# Autodesk Inventor assembly: Ensamble del Sistema de Balanceo
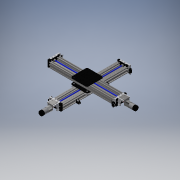
[picture p0: Inventor's stored thumbnail of the model, 180x180]
Saved by Autodesk Inventor 2018.3 (Build 223284000, 284)
## iProperties
Created: 2020-12-03
Part Number: Ensamble del Sistema de Balanceo
Material: Genérico
Description: STEP AP203
Document SubType Name: Assembly
Designer: SERGIO ROMO
Sending System: SolidWorks 2019
Preprocessor: SwSTEP 2.0
Title: Ensamble del Arreglo.STEP
Revision Number: ANY
## Documents named in this file (17)
- C:\Users\SERGIO ROMO\Documents\GitHub\RemBot\CAD\Balanceo de masa\Inventor\Ensamble del Sistema de Balanceo.iam
- C:\Users\SERGIO ROMO\Documents\GitHub\RemBot\CAD\Balanceo de masa\Inventor\C-Beam Actuator Lineal 500mm (Sin motor, sin carrito).ipt
- C:\Users\SERGIO ROMO\Documents\GitHub\RemBot\CAD\Balanceo de masa\Inventor\XLarge C-Beam Gantry Kit.iam
- C:\Users\SERGIO ROMO\Documents\GitHub\RemBot\CAD\Balanceo de masa\Inventor\Clavo.ipt
- C:\Users\SERGIO ROMO\Documents\GitHub\RemBot\CAD\Balanceo de masa\Inventor\Gearmotor_37D_19a1.ipt
- C:\Users\SERGIO ROMO\Documents\GitHub\RemBot\CAD\Balanceo de masa\Inventor\Impresion3D.ipt
- C:\Users\SERGIO ROMO\Documents\GitHub\RemBot\CAD\Balanceo de masa\Inventor\C-Beam Gantry Plate XLarge.step.ipt
- C:\Users\SERGIO ROMO\Documents\GitHub\RemBot\CAD\Balanceo de masa\Inventor\Bracket Inventor.ipt
- C:\Users\SERGIO ROMO\Documents\GitHub\RemBot\CAD\Balanceo de masa\Inventor\KW8-2.ipt
- C:\Users\SERGIO ROMO\Documents\GitHub\RemBot\CAD\Balanceo de masa\Inventor\Impresion3D sin Bracket.ipt
- C:\Users\SERGIO ROMO\Documents\GitHub\RemBot\CAD\Balanceo de masa\Inventor\Clavo de Arriba.ipt
- C:\Users\SERGIO ROMO\Documents\GitHub\RemBot\CAD\Balanceo de masa\Inventor\Tornillo final de carrera.ipt
- C:\Users\SERGIO ROMO\Documents\GitHub\RemBot\CAD\Balanceo de masa\Inventor\Triangulo.ipt
- C:\Users\SERGIO ROMO\Documents\GitHub\RemBot\CAD\Balanceo de masa\Inventor\TornilloM6.ipt
- C:\Users\SERGIO ROMO\Documents\GitHub\RemBot\CAD\Balanceo de masa\Inventor\Tuerca para tornilloM6.ipt
- C:\Users\SERGIO ROMO\Documents\GitHub\RemBot\CAD\Balanceo de masa\Inventor\Tornillo para Bracket.ipt
- C:\Users\SERGIO ROMO\Documents\GitHub\RemBot\CAD\Balanceo de masa\Inventor\Tornillo para Motor Pololu.ipt
## Components (68 placed, 21 different names)
1. C-Beam Actuator Lineal 500mm (Sin motor, sin carrito)_1 — Coincidencia:6, Coincidencia:7, Coincidencia:8, Coincidencia:39, Coincidencia:41, Coincidencia:42, Coincidencia:45
2. XLarge C-Beam Gantry Kit_2 [sub-assembly] — Rígido:1
3. Clavo_8
4. Clavo_9
5. Gearmotor_37D_19a1_10 — Coincidencia:6
6. Gearmotor_37D_19a1_22
7. Impresion3D_28 — Coincidencia:1, Coincidencia:4, Coincidencia:15, Coincidencia:16, Coincidencia:28, Coincidencia:29, Coincidencia:30, Coincidencia:31, Coincidencia:83, Coincidencia:84
8. C-Beam Actuator Lineal 500mm (Sin motor, sin carrito):2 — Rígido:1, Coincidencia:2, Coincidencia:9, Coincidencia:10
9. C-Beam Gantry Plate XLarge.step:1
10. Bracket Inventor:1 — Coincidencia:1, Coincidencia:83, Coincidencia:84, Coincidencia:106, Coincidencia:107, Coincidencia:108, Coincidencia:109, Coincidencia:110, Coincidencia:111, Coincidencia:112, Coincidencia:113, Coincidencia:134, Coincidencia:135, Coincidencia:136, Coincidencia:137, Coincidencia:138, Coincidencia:139, Coincidencia:140, Coincidencia:141, Coincidencia:142, Coincidencia:143, Coincidencia:144, Coincidencia:145
11. Bracket Inventor:2 — Coincidencia:3, Coincidencia:11, Coincidencia:12, Coincidencia:85, Coincidencia:114, Coincidencia:115, Coincidencia:116, Coincidencia:117, Coincidencia:118, Coincidencia:119, Coincidencia:120, Coincidencia:121, Coincidencia:122, Coincidencia:123, Coincidencia:124, Coincidencia:125, Coincidencia:126, Coincidencia:127, Coincidencia:128, Coincidencia:129, Coincidencia:130, Coincidencia:131, Coincidencia:132, Coincidencia:133
12. Impresion3D:2 — Coincidencia:2, Coincidencia:3, Coincidencia:5, Coincidencia:11, Coincidencia:12, Coincidencia:13, Coincidencia:14, Coincidencia:24, Coincidencia:25, Coincidencia:26, Coincidencia:27, Coincidencia:85, Coincidencia:90, Coincidencia:91, Coincidencia:92, Coincidencia:93
13. KW8-2:1 — Coincidencia:4
14. KW8-2:2 — Coincidencia:5
15. KW8-2:3
16. KW8-2:4
17. Impresion3D sin Bracket:1 — Coincidencia:7, Coincidencia:8, Coincidencia:17, Coincidencia:18, Coincidencia:19, Coincidencia:86, Coincidencia:87, Coincidencia:88, Coincidencia:89
18. Impresion3D sin Bracket:2 — Coincidencia:9, Coincidencia:10, Coincidencia:20, Coincidencia:21, Coincidencia:22, Coincidencia:23, Coincidencia:94, Coincidencia:95, Coincidencia:96, Coincidencia:97
19. Clavo:3 — Coincidencia:13
20. Clavo:4 — Coincidencia:14
21. Clavo de Arriba:1 — Coincidencia:15
22. Clavo de Arriba:2 — Coincidencia:16
23. Clavo de Arriba:3 — Coincidencia:17
24. Clavo de Arriba:4 — Coincidencia:18, Coincidencia:19
25. Clavo de Arriba:5 — Coincidencia:21, Coincidencia:23
26. Clavo de Arriba:6 — Coincidencia:20, Coincidencia:22
27. Clavo de Arriba:7 — Coincidencia:24, Coincidencia:25
28. Clavo de Arriba:8 — Coincidencia:26, Coincidencia:27
29. Tornillo final de carrera:1 — Coincidencia:28, Coincidencia:30
30. Tornillo final de carrera:2 — Coincidencia:29, Coincidencia:31
31. Triangulo:1 — Coincidencia:41, Coincidencia:102, Coincidencia:104
32. Triangulo:2 — Coincidencia:42, Coincidencia:98, Coincidencia:100
33. Triangulo:3 — Coincidencia:39, Coincidencia:103, Coincidencia:105
34. Triangulo:4 — Coincidencia:45, Coincidencia:99, Coincidencia:101
35. Tornillo final de carrera:3 — Coincidencia:86, Coincidencia:88
36. Tornillo final de carrera:4 — Coincidencia:87, Coincidencia:89
37. Tornillo final de carrera:5 — Coincidencia:90, Coincidencia:92
38. Tornillo final de carrera:6 — Coincidencia:91, Coincidencia:93
39. Tornillo final de carrera:7 — Coincidencia:94, Coincidencia:96
40. Tornillo final de carrera:8 — Coincidencia:95, Coincidencia:97
41. TornilloM6:5 — Coincidencia:98
42. TornilloM6:6 — Coincidencia:99
43. Tuerca para tornilloM6:5 — Coincidencia:100
44. Tuerca para tornilloM6:6 — Coincidencia:101
45. TornilloM6:7 — Coincidencia:102
46. TornilloM6:8 — Coincidencia:103
47. Tuerca para tornilloM6:7 — Coincidencia:105
48. Tuerca para tornilloM6:8 — Coincidencia:104
49. Tornillo para Bracket:1 — Coincidencia:107, Coincidencia:111
50. Tornillo para Bracket:2 — Coincidencia:108, Coincidencia:112
51. Tornillo para Bracket:3 — Coincidencia:109, Coincidencia:110
52. Tornillo para Bracket:4 — Coincidencia:106, Coincidencia:113
53. Tornillo para Bracket:5 — Coincidencia:116, Coincidencia:121
54. Tornillo para Bracket:6 — Coincidencia:115, Coincidencia:118
55. Tornillo para Bracket:7 — Coincidencia:117, Coincidencia:120
56. Tornillo para Bracket:8 — Coincidencia:114, Coincidencia:119
57. Tornillo para Motor Pololu:1 — Coincidencia:127, Coincidencia:130
58. Tornillo para Motor Pololu:2 — Coincidencia:126, Coincidencia:128
59. Tornillo para Motor Pololu:3 — Coincidencia:124, Coincidencia:132
60. Tornillo para Motor Pololu:4 — Coincidencia:123, Coincidencia:131
61. Tornillo para Motor Pololu:5 — Coincidencia:125, Coincidencia:129
62. Tornillo para Motor Pololu:6 — Coincidencia:122, Coincidencia:133
63. Tornillo para Motor Pololu:7 — Coincidencia:138, Coincidencia:144
64. Tornillo para Motor Pololu:8 — Coincidencia:137, Coincidencia:143
65. Tornillo para Motor Pololu:9 — Coincidencia:136, Coincidencia:145
66. Tornillo para Motor Pololu:10 — Coincidencia:134, Coincidencia:141
67. Tornillo para Motor Pololu:11 — Coincidencia:135, Coincidencia:140
68. Tornillo para Motor Pololu:12 — Coincidencia:139, Coincidencia:142
## Relationships (99: Mate 98, WeldJoint 1)
- Rígido:1 [WeldJoint]: XLarge C-Beam Gantry Kit_2 ↔ C-Beam Actuator Lineal 500mm (Sin motor, sin carrito):2
- Coincidencia:1 [Mate]: Impresion3D_28 ↔ Bracket Inventor:1
- Coincidencia:2 [Mate]: C-Beam Actuator Lineal 500mm (Sin motor, sin carrito):2 ↔ Impresion3D:2
- Coincidencia:3 [Mate]: Bracket Inventor:2 ↔ Impresion3D:2
- Coincidencia:4 [Mate]: Impresion3D_28 ↔ KW8-2:1
- Coincidencia:5 [Mate]: Impresion3D:2 ↔ KW8-2:2
- Coincidencia:6 [Mate]: C-Beam Actuator Lineal 500mm (Sin motor, sin carrito)_1 ↔ Gearmotor_37D_19a1_10
- Coincidencia:7 [Mate]: C-Beam Actuator Lineal 500mm (Sin motor, sin carrito)_1 ↔ Impresion3D sin Bracket:1
- Coincidencia:8 [Mate]: C-Beam Actuator Lineal 500mm (Sin motor, sin carrito)_1 ↔ Impresion3D sin Bracket:1
- Coincidencia:9 [Mate]: C-Beam Actuator Lineal 500mm (Sin motor, sin carrito):2 ↔ Impresion3D sin Bracket:2
- Coincidencia:10 [Mate]: C-Beam Actuator Lineal 500mm (Sin motor, sin carrito):2 ↔ Impresion3D sin Bracket:2
- Coincidencia:11 [Mate]: Bracket Inventor:2 ↔ Impresion3D:2
- Coincidencia:12 [Mate]: Bracket Inventor:2 ↔ Impresion3D:2
- Coincidencia:13 [Mate]: Impresion3D:2 ↔ Clavo:3
- Coincidencia:14 [Mate]: Impresion3D:2 ↔ Clavo:4
- Coincidencia:15 [Mate]: Impresion3D_28 ↔ Clavo de Arriba:1
- Coincidencia:16 [Mate]: Impresion3D_28 ↔ Clavo de Arriba:2
- Coincidencia:17 [Mate]: Impresion3D sin Bracket:1 ↔ Clavo de Arriba:3
- Coincidencia:18 [Mate]: Impresion3D sin Bracket:1 ↔ Clavo de Arriba:4
- Coincidencia:19 [Mate]: Impresion3D sin Bracket:1 ↔ Clavo de Arriba:4
- Coincidencia:20 [Mate]: Impresion3D sin Bracket:2 ↔ Clavo de Arriba:6
- Coincidencia:21 [Mate]: Impresion3D sin Bracket:2 ↔ Clavo de Arriba:5
- Coincidencia:22 [Mate]: Impresion3D sin Bracket:2 ↔ Clavo de Arriba:6
- Coincidencia:23 [Mate]: Impresion3D sin Bracket:2 ↔ Clavo de Arriba:5
- Coincidencia:24 [Mate]: Impresion3D:2 ↔ Clavo de Arriba:7
- Coincidencia:25 [Mate]: Impresion3D:2 ↔ Clavo de Arriba:7
- Coincidencia:26 [Mate]: Impresion3D:2 ↔ Clavo de Arriba:8
- Coincidencia:27 [Mate]: Impresion3D:2 ↔ Clavo de Arriba:8
- Coincidencia:28 [Mate]: Impresion3D_28 ↔ Tornillo final de carrera:1
- Coincidencia:29 [Mate]: Impresion3D_28 ↔ Tornillo final de carrera:2
- Coincidencia:30 [Mate]: Impresion3D_28 ↔ Tornillo final de carrera:1
- Coincidencia:31 [Mate]: Impresion3D_28 ↔ Tornillo final de carrera:2
- Coincidencia:39 [Mate]: C-Beam Actuator Lineal 500mm (Sin motor, sin carrito)_1 ↔ Triangulo:3
- Coincidencia:41 [Mate]: C-Beam Actuator Lineal 500mm (Sin motor, sin carrito)_1 ↔ Triangulo:1
- Coincidencia:42 [Mate]: C-Beam Actuator Lineal 500mm (Sin motor, sin carrito)_1 ↔ Triangulo:2
- Coincidencia:45 [Mate]: C-Beam Actuator Lineal 500mm (Sin motor, sin carrito)_1 ↔ Triangulo:4
- Coincidencia:83 [Mate]: Impresion3D_28 ↔ Bracket Inventor:1
- Coincidencia:84 [Mate]: Impresion3D_28 ↔ Bracket Inventor:1
- Coincidencia:85 [Mate]: Bracket Inventor:2 ↔ Impresion3D:2
- Coincidencia:86 [Mate]: Impresion3D sin Bracket:1 ↔ Tornillo final de carrera:3
- Coincidencia:87 [Mate]: Impresion3D sin Bracket:1 ↔ Tornillo final de carrera:4
- Coincidencia:88 [Mate]: Impresion3D sin Bracket:1 ↔ Tornillo final de carrera:3
- Coincidencia:89 [Mate]: Impresion3D sin Bracket:1 ↔ Tornillo final de carrera:4
- Coincidencia:90 [Mate]: Impresion3D:2 ↔ Tornillo final de carrera:5
- Coincidencia:91 [Mate]: Impresion3D:2 ↔ Tornillo final de carrera:6
- Coincidencia:92 [Mate]: Impresion3D:2 ↔ Tornillo final de carrera:5
- Coincidencia:93 [Mate]: Impresion3D:2 ↔ Tornillo final de carrera:6
- Coincidencia:94 [Mate]: Impresion3D sin Bracket:2 ↔ Tornillo final de carrera:7
- Coincidencia:95 [Mate]: Impresion3D sin Bracket:2 ↔ Tornillo final de carrera:8
- Coincidencia:96 [Mate]: Impresion3D sin Bracket:2 ↔ Tornillo final de carrera:7
- Coincidencia:97 [Mate]: Impresion3D sin Bracket:2 ↔ Tornillo final de carrera:8
- Coincidencia:98 [Mate]: Triangulo:2 ↔ TornilloM6:5
- Coincidencia:99 [Mate]: Triangulo:4 ↔ TornilloM6:6
- Coincidencia:100 [Mate]: Triangulo:2 ↔ Tuerca para tornilloM6:5
- Coincidencia:101 [Mate]: Triangulo:4 ↔ Tuerca para tornilloM6:6
- Coincidencia:102 [Mate]: Triangulo:1 ↔ TornilloM6:7
- Coincidencia:103 [Mate]: Triangulo:3 ↔ TornilloM6:8
- Coincidencia:104 [Mate]: Triangulo:1 ↔ Tuerca para tornilloM6:8
- Coincidencia:105 [Mate]: Triangulo:3 ↔ Tuerca para tornilloM6:7
- Coincidencia:106 [Mate]: Bracket Inventor:1 ↔ Tornillo para Bracket:4
- Coincidencia:107 [Mate]: Bracket Inventor:1 ↔ Tornillo para Bracket:1
- Coincidencia:108 [Mate]: Bracket Inventor:1 ↔ Tornillo para Bracket:2
- Coincidencia:109 [Mate]: Bracket Inventor:1 ↔ Tornillo para Bracket:3
- Coincidencia:110 [Mate]: Bracket Inventor:1 ↔ Tornillo para Bracket:3
- Coincidencia:111 [Mate]: Bracket Inventor:1 ↔ Tornillo para Bracket:1
- Coincidencia:112 [Mate]: Bracket Inventor:1 ↔ Tornillo para Bracket:2
- Coincidencia:113 [Mate]: Bracket Inventor:1 ↔ Tornillo para Bracket:4
- Coincidencia:114 [Mate]: Bracket Inventor:2 ↔ Tornillo para Bracket:8
- Coincidencia:115 [Mate]: Bracket Inventor:2 ↔ Tornillo para Bracket:6
- Coincidencia:116 [Mate]: Bracket Inventor:2 ↔ Tornillo para Bracket:5
- Coincidencia:117 [Mate]: Bracket Inventor:2 ↔ Tornillo para Bracket:7
- Coincidencia:118 [Mate]: Bracket Inventor:2 ↔ Tornillo para Bracket:6
- Coincidencia:119 [Mate]: Bracket Inventor:2 ↔ Tornillo para Bracket:8
- Coincidencia:120 [Mate]: Bracket Inventor:2 ↔ Tornillo para Bracket:7
- Coincidencia:121 [Mate]: Bracket Inventor:2 ↔ Tornillo para Bracket:5
- Coincidencia:122 [Mate]: Bracket Inventor:2 ↔ Tornillo para Motor Pololu:6
- Coincidencia:123 [Mate]: Bracket Inventor:2 ↔ Tornillo para Motor Pololu:4
- Coincidencia:124 [Mate]: Bracket Inventor:2 ↔ Tornillo para Motor Pololu:3
- Coincidencia:125 [Mate]: Bracket Inventor:2 ↔ Tornillo para Motor Pololu:5
- Coincidencia:126 [Mate]: Bracket Inventor:2 ↔ Tornillo para Motor Pololu:2
- Coincidencia:127 [Mate]: Bracket Inventor:2 ↔ Tornillo para Motor Pololu:1
- Coincidencia:128 [Mate]: Bracket Inventor:2 ↔ Tornillo para Motor Pololu:2
- Coincidencia:129 [Mate]: Bracket Inventor:2 ↔ Tornillo para Motor Pololu:5
- Coincidencia:130 [Mate]: Bracket Inventor:2 ↔ Tornillo para Motor Pololu:1
- Coincidencia:131 [Mate]: Bracket Inventor:2 ↔ Tornillo para Motor Pololu:4
- Coincidencia:132 [Mate]: Bracket Inventor:2 ↔ Tornillo para Motor Pololu:3
- Coincidencia:133 [Mate]: Bracket Inventor:2 ↔ Tornillo para Motor Pololu:6
- Coincidencia:134 [Mate]: Bracket Inventor:1 ↔ Tornillo para Motor Pololu:10
- Coincidencia:135 [Mate]: Bracket Inventor:1 ↔ Tornillo para Motor Pololu:11
- Coincidencia:136 [Mate]: Bracket Inventor:1 ↔ Tornillo para Motor Pololu:9
- Coincidencia:137 [Mate]: Bracket Inventor:1 ↔ Tornillo para Motor Pololu:8
- Coincidencia:138 [Mate]: Bracket Inventor:1 ↔ Tornillo para Motor Pololu:7
- Coincidencia:139 [Mate]: Bracket Inventor:1 ↔ Tornillo para Motor Pololu:12
- Coincidencia:140 [Mate]: Bracket Inventor:1 ↔ Tornillo para Motor Pololu:11
- Coincidencia:141 [Mate]: Bracket Inventor:1 ↔ Tornillo para Motor Pololu:10
- Coincidencia:142 [Mate]: Bracket Inventor:1 ↔ Tornillo para Motor Pololu:12
- Coincidencia:143 [Mate]: Bracket Inventor:1 ↔ Tornillo para Motor Pololu:8
- Coincidencia:144 [Mate]: Bracket Inventor:1 ↔ Tornillo para Motor Pololu:7
- Coincidencia:145 [Mate]: Bracket Inventor:1 ↔ Tornillo para Motor Pololu:9
